# Autodesk Inventor assembly: HC-05+module
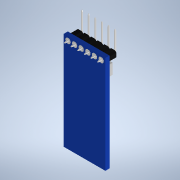
[picture p0: Inventor's stored thumbnail of the model, 180x180]
Saved by Autodesk Inventor 2021 (Build 250183000, 183)
## iProperties
Created: 2021-07-24
Part Number: HC-05+module
Document SubType Name: Assembly
Designer: ermoz
Author: ermoz
## Documents named in this file (4)
- D:\Moje Wyczyny\My_Poor_Projects\Sneak100_MiniSumo\minisumo-sneak100\mechanics\ElectricElements\HC-05_module.iam
- D:\Moje Wyczyny\My_Poor_Projects\Sneak100_MiniSumo\minisumo-sneak100\mechanics\ElectricElements\ZS-040.ipt
- D:\Moje Wyczyny\My_Poor_Projects\Sneak100_MiniSumo\minisumo-sneak100\mechanics\ElectricElements\HC-05.ipt
- D:\Moje Wyczyny\My_Poor_Projects\Sneak100_MiniSumo\minisumo-sneak100\mechanics\ElectricElements\MaleHeaderPin_1x6_90.iam
## Components (3 placed, 3 different names)
1. ZS-040:1 — Mate:1, Flush:1, Flush:2, Mate:2, Tangent:1, Tangent:2, Tangent:3
2. HC-05:1 — Mate:1, Flush:1, Flush:2
3. MaleHeaderPin_1x6_90:1 [sub-assembly] — Mate:2, Tangent:1, Tangent:2, Tangent:3
## Relationships (7: Tangent 3, Mate 2, Flush 2)
- Mate:1: ZS-040:1 ↔ HC-05:1
- Flush:1 (0.5 mm): ZS-040:1 ↔ HC-05:1
- Flush:2 (1.5 mm): ZS-040:1 ↔ HC-05:1
- Mate:2: ZS-040:1 ↔ MaleHeaderPin_1x6_90:1
- Tangent:1 (-0.3 mm): ZS-040:1 ↔ MaleHeaderPin_1x6_90:1
- Tangent:2 (-0.3 mm): ZS-040:1 ↔ MaleHeaderPin_1x6_90:1
- Tangent:3 (-0.3 mm): ZS-040:1 ↔ MaleHeaderPin_1x6_90:1
